# Autodesk Inventor assembly: FLEX_KURT D688
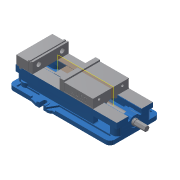
[picture p0: Inventor's stored thumbnail of the model, 180x180]
Saved by Autodesk Inventor 2021.4 (Build 254397000, 397)
## iProperties
Created: 2022-03-02
Part Number: FLEX_KURT D688
Document SubType Name: Assembly
Designer: rodar
Author: rodar
## Documents named in this file (3)
- C:\Users\rodar\OneDrive\Desktop\INVENTOR\UVG\EQUIPO TALLER\WORK HOLDING\KURT\FLEX_KURT D688.iam
- C:\Users\rodar\OneDrive\Desktop\INVENTOR\UVG\EQUIPO TALLER\WORK HOLDING\KURT\D_KURT D688 BASE.ipt
- C:\Users\rodar\OneDrive\Desktop\INVENTOR\UVG\EQUIPO TALLER\WORK HOLDING\KURT\D_KURT D688 JAW.ipt
## Components (2 placed, 2 different names)
1. D_KURT D688 BASE:1 — Flush:1, Flush:2
2. D_KURT D688 JAW:1 — Flush:1, Flush:2
## Relationships (2: Flush 2)
- Flush:1: D_KURT D688 BASE:1 ↔ D_KURT D688 JAW:1
- Flush:2: D_KURT D688 BASE:1 ↔ D_KURT D688 JAW:1
